# Autodesk Inventor assembly: RT_MAIN_A_001
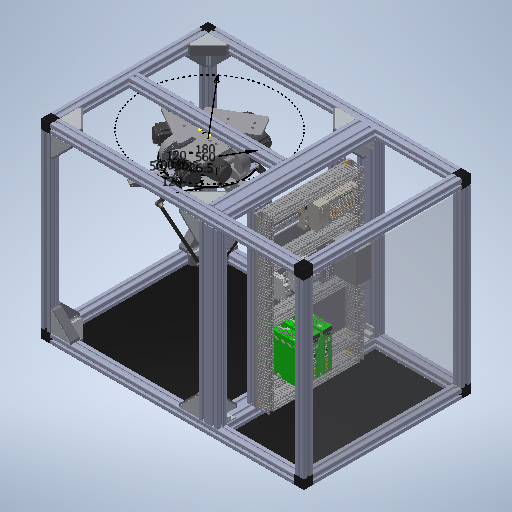
[picture p0: Inventor's stored thumbnail of the model, 512x512]
Saved by Autodesk Inventor 2025.3 (Build 293356000, 356)
## iProperties
Created: 2026-05-15
Part Number: RT_MAIN_A_001
Document SubType Name: Assembly
Designer: louis
Mass: 34530.7 g
Surface Area: 112620 cm^2
Volume: 12343.4 cm^3
Density: 2.7975 g/cm^3
Author: louis
## Documents named in this file (6)
- C:\Users\louis\OneDrive\Desktop\R_Trident\02_CAD\05_Top_Assembly\RT_MAIN_A_001.iam
- C:\Users\louis\OneDrive\Desktop\R_Trident\02_CAD\04_Subassemblies\RT_FRM_A_003_FrameV5.iam
- C:\Users\louis\OneDrive\Desktop\R_Trident\02_CAD\04_Subassemblies\RT_ELE_001_ElectricalMainPlate_V0.2.iam
- C:\Users\louis\OneDrive\Desktop\R_Trident\02_CAD\04_Subassemblies\RT_FRM_A_002_Dynamics.iam
- C:\Users\louis\OneDrive\Desktop\R_Trident\02_CAD\04_Subassemblies\TempPart1.ipt
- C:\Users\louis\OneDrive\Desktop\R_Trident\02_CAD\04_Subassemblies\RT_ARM_A_007_Capstan-Drive.iam
## Components (7 placed, 5 different names)
1. RT_FRM_A_003_FrameV5:1 [sub-assembly] — Mate:1, Mate:2, Mate:3, Mate:4, Mate:5, Mate:6, Flush:8, Mate:16
2. RT_ELE_001_ElectricalMainPlate_V0.2:1 [sub-assembly] — Mate:4, Mate:5
3. RT_FRM_A_002_Dynamics:1 [sub-assembly] — Mate:6, Flush:8
4. TempPart1:1 — Mate:7, Mate:8, Mate:9, Mate:10, Mate:11, Mate:12, Mate:13, Mate:14, Mate:15, Mate:16
5. RT_ARM_A_007_Capstan-Drive:1 [sub-assembly] — Mate:7, Mate:8, Mate:14
6. RT_ARM_A_007_Capstan-Drive:2 [sub-assembly] — Mate:9, Mate:10, Mate:13
7. RT_ARM_A_007_Capstan-Drive:3 [sub-assembly] — Mate:11, Mate:12, Mate:15
## Relationships (17: Mate 16, Flush 1)
- Mate:1: RT_FRM_A_003_FrameV5:1
- Mate:2: RT_FRM_A_003_FrameV5:1
- Mate:3: RT_FRM_A_003_FrameV5:1
- Mate:4: RT_FRM_A_003_FrameV5:1 ↔ RT_ELE_001_ElectricalMainPlate_V0.2:1
- Mate:5: RT_FRM_A_003_FrameV5:1 ↔ RT_ELE_001_ElectricalMainPlate_V0.2:1
- Mate:6: RT_FRM_A_003_FrameV5:1 ↔ RT_FRM_A_002_Dynamics:1
- Flush:8: RT_FRM_A_003_FrameV5:1 ↔ RT_FRM_A_002_Dynamics:1
- Mate:7: TempPart1:1 ↔ RT_ARM_A_007_Capstan-Drive:1
- Mate:8: TempPart1:1 ↔ RT_ARM_A_007_Capstan-Drive:1
- Mate:9: TempPart1:1 ↔ RT_ARM_A_007_Capstan-Drive:2
- Mate:10: TempPart1:1 ↔ RT_ARM_A_007_Capstan-Drive:2
- Mate:11: TempPart1:1 ↔ RT_ARM_A_007_Capstan-Drive:3
- Mate:12: TempPart1:1 ↔ RT_ARM_A_007_Capstan-Drive:3
- Mate:13: TempPart1:1 ↔ RT_ARM_A_007_Capstan-Drive:2
- Mate:14: TempPart1:1 ↔ RT_ARM_A_007_Capstan-Drive:1
- Mate:15: TempPart1:1 ↔ RT_ARM_A_007_Capstan-Drive:3
- Mate:16 (100 mm): RT_FRM_A_003_FrameV5:1 ↔ TempPart1:1
